# Autodesk Inventor assembly: 000-base_wheel-v1
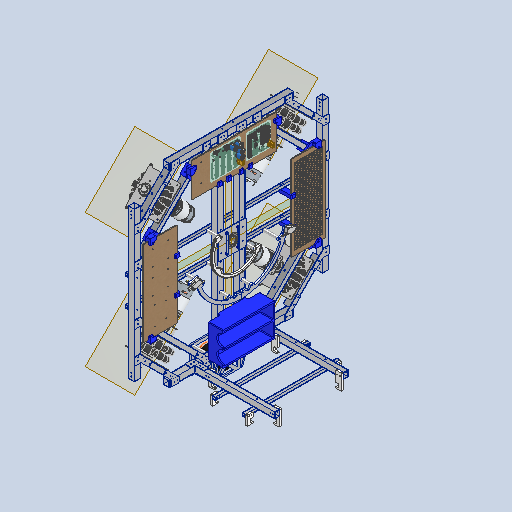
[picture p0: Inventor's stored thumbnail of the model, 512x512]
Saved by Autodesk Inventor 2025.2 (Build 292293000, 293)
## iProperties
Created: 2025-01-06
Part Number: 000-base_wheel-v1
Document SubType Name: Assembly
Designer: haruy
Mass: 4431.15 g
Surface Area: 15153.5 cm^2
Volume: 1600.59 cm^3
Density: 2.76846 g/cm^3
Author: haruy
## Documents named in this file (72)
- C:\Users\haruy\Documents\ロボコン\NHK2025\cad\nagahisa\base_weel\000-base_wheel-v1.iam
- C:\Users\haruy\Documents\ロボコン\NHK2025\cad\nagahisa\base_weel\base_weel-v2-ASP-Base.ipt
- C:\Users\haruy\Documents\ロボコン\NHK2025\cad\nagahisa\base_weel\base_weel-v2-Plate-1.ipt
- C:\Users\haruy\Documents\ロボコン\NHK2025\cad\nagahisa\base_weel\C-FL6904ZZ.ipt
- C:\Users\haruy\Documents\ロボコン\NHK2025\cad\nagahisa\base_weel\base_weel-v1-Shaft-spesa-1.ipt
- C:\Users\haruy\Documents\ロボコン\NHK2025\cad\nagahisa\base_weel\base_weel-v2-Plate-2.ipt
- C:\Users\haruy\Documents\ロボコン\NHK2025\cad\nagahisa\base_weel\takagi_weel\Workspaces\作業スペース\takagi\omuni_wheel_ver3.0\parts\omu_al_jo_1.ipt
- C:\Users\haruy\Documents\ロボコン\NHK2025\cad\nagahisa\base_weel\takagi_weel\Workspaces\作業スペース\takagi\omuni_wheel_ver3.0\parts\omu_al_jo_3.ipt
- C:\Users\haruy\Documents\ロボコン\NHK2025\cad\nagahisa\base_weel\takagi_weel\Workspaces\作業スペース\takagi\omuni_wheel_ver3.0\parts\frequently used parts\モーター\RS775\rs775_4.iam
- C:\Users\haruy\Documents\ロボコン\NHK2025\cad\nagahisa\base_weel\takagi_weel\Workspaces\作業スペース\takagi\omuni_wheel_ver3.0\parts\frequently used parts\セットカラー\SSCSP12-10\SSCSP12-10.iam
- C:\Users\haruy\Documents\ロボコン\NHK2025\cad\nagahisa\base_weel\takagi_weel\Workspaces\作業スペース\takagi\omuni_wheel_ver3.0\parts\omu_al_jo_2.ipt
- C:\Users\haruy\Documents\ロボコン\NHK2025\cad\nagahisa\base_weel\takagi_weel\Workspaces\作業スペース\takagi\omuni_wheel_ver3.0\parts\omu_sh_jo_2.ipt
- C:\Users\haruy\Documents\ロボコン\NHK2025\cad\nagahisa\base_weel\takagi_weel\Workspaces\作業スペース\takagi\omuni_wheel_ver3.0\parts\omu_sh_jo_3.ipt
- C:\Users\haruy\Documents\ロボコン\NHK2025\cad\nagahisa\base_weel\takagi_weel\Workspaces\作業スペース\takagi\omuni_wheel_ver3.0\parts\frequently used parts\ベアリング\B6201ZZNR\bearingB6201ZZNR.ipt
- C:\Users\haruy\Documents\ロボコン\NHK2025\cad\nagahisa\base_weel\takagi_weel\Workspaces\作業スペース\takagi\omuni_wheel_ver3.0\parts\frequently used parts\タイヤ\omni wheel\100mm wheel\100mm omuniwheel_MIR1.iam
- C:\Users\haruy\Documents\ロボコン\NHK2025\cad\nagahisa\base_weel\base_weel-v1-Shaft-spesa-2.ipt
- C:\Users\haruy\Documents\ロボコン\NHK2025\cad\nagahisa\base_weel\000-base_wheel-v1\デザイン アクセラレータ\平歯車1.iam
- C:\Users\haruy\Documents\ロボコン\NHK2025\cad\nagahisa\base_weel\base_weel-v1-Shaft-spesa-3.ipt
- C:\Users\haruy\Documents\ロボコン\NHK2025\cad\nagahisa\base_weel\takagi_weel\Workspaces\作業スペース\takagi\omuni_wheel_ver3.0\parts\omu_al_jo_1_MIR2.ipt
- C:\Users\haruy\Documents\ロボコン\NHK2025\cad\nagahisa\base_weel\takagi_weel\Workspaces\作業スペース\takagi\omuni_wheel_ver3.0\parts\omu_al_jo_3_MIR2.ipt
- C:\Users\haruy\Documents\ロボコン\NHK2025\cad\nagahisa\base_weel\takagi_weel\Workspaces\作業スペース\takagi\omuni_wheel_ver3.0\parts\frequently used parts\モーター\RS775\rs775_4_MIR2.iam
- C:\Users\haruy\Documents\ロボコン\NHK2025\cad\nagahisa\base_weel\takagi_weel\Workspaces\作業スペース\takagi\omuni_wheel_ver3.0\parts\frequently used parts\セットカラー\SSCSP12-10\SSCSP12-10_MIR2.iam
- C:\Users\haruy\Documents\ロボコン\NHK2025\cad\nagahisa\base_weel\takagi_weel\Workspaces\作業スペース\takagi\omuni_wheel_ver3.0\parts\omu_al_jo_2_MIR2.ipt
- C:\Users\haruy\Documents\ロボコン\NHK2025\cad\nagahisa\base_weel\takagi_weel\Workspaces\作業スペース\takagi\omuni_wheel_ver3.0\parts\omu_sh_jo_2_MIR2.ipt
- C:\Users\haruy\Documents\ロボコン\NHK2025\cad\nagahisa\base_weel\takagi_weel\Workspaces\作業スペース\takagi\omuni_wheel_ver3.0\parts\omu_sh_jo_3_MIR2.ipt
- C:\Users\haruy\Documents\ロボコン\NHK2025\cad\nagahisa\base_weel\takagi_weel\Workspaces\作業スペース\takagi\omuni_wheel_ver3.0\parts\frequently used parts\ベアリング\B6201ZZNR\bearingB6201ZZNR_MIR2.ipt
- C:\Users\haruy\Documents\ロボコン\NHK2025\cad\nagahisa\base_weel\takagi_weel\Workspaces\作業スペース\takagi\omuni_wheel_ver3.0\parts\frequently used parts\タイヤ\omni wheel\100mm wheel\100mm omuniwheel_MIR1_MIR.iam
- C:\Users\haruy\Documents\ロボコン\NHK2025\cad\nagahisa\base_weel\takagi_weel\Workspaces\作業スペース\takagi\omuni_wheel_ver3.0\parts\omu_al_jo_1_MIR3.ipt
- C:\Users\haruy\Documents\ロボコン\NHK2025\cad\nagahisa\base_weel\takagi_weel\Workspaces\作業スペース\takagi\omuni_wheel_ver3.0\parts\omu_al_jo_3_MIR3.ipt
- C:\Users\haruy\Documents\ロボコン\NHK2025\cad\nagahisa\base_weel\takagi_weel\Workspaces\作業スペース\takagi\omuni_wheel_ver3.0\parts\frequently used parts\モーター\RS775\rs775_4_MIR3.iam
- C:\Users\haruy\Documents\ロボコン\NHK2025\cad\nagahisa\base_weel\takagi_weel\Workspaces\作業スペース\takagi\omuni_wheel_ver3.0\parts\frequently used parts\セットカラー\SSCSP12-10\SSCSP12-10_MIR3.iam
- C:\Users\haruy\Documents\ロボコン\NHK2025\cad\nagahisa\base_weel\takagi_weel\Workspaces\作業スペース\takagi\omuni_wheel_ver3.0\parts\omu_al_jo_2_MIR3.ipt
- C:\Users\haruy\Documents\ロボコン\NHK2025\cad\nagahisa\base_weel\takagi_weel\Workspaces\作業スペース\takagi\omuni_wheel_ver3.0\parts\omu_sh_jo_2_MIR3.ipt
- C:\Users\haruy\Documents\ロボコン\NHK2025\cad\nagahisa\base_weel\takagi_weel\Workspaces\作業スペース\takagi\omuni_wheel_ver3.0\parts\omu_sh_jo_3_MIR3.ipt
- C:\Users\haruy\Documents\ロボコン\NHK2025\cad\nagahisa\base_weel\takagi_weel\Workspaces\作業スペース\takagi\omuni_wheel_ver3.0\parts\frequently used parts\ベアリング\B6201ZZNR\bearingB6201ZZNR_MIR3.ipt
- C:\Users\haruy\Documents\ロボコン\NHK2025\cad\nagahisa\base_weel\takagi_weel\Workspaces\作業スペース\takagi\omuni_wheel_ver3.0\parts\frequently used parts\タイヤ\omni wheel\100mm wheel\100mm omuniwheel_MIR1_MIR1.iam
- C:\Users\haruy\Documents\ロボコン\NHK2025\cad\nagahisa\base_weel\takagi_weel\Workspaces\作業スペース\takagi\omuni_wheel_ver3.0\parts\omu_al_jo_1_MIR2_MIR.ipt
- C:\Users\haruy\Documents\ロボコン\NHK2025\cad\nagahisa\base_weel\takagi_weel\Workspaces\作業スペース\takagi\omuni_wheel_ver3.0\parts\omu_al_jo_3_MIR2_MIR.ipt
- C:\Users\haruy\Documents\ロボコン\NHK2025\cad\nagahisa\base_weel\takagi_weel\Workspaces\作業スペース\takagi\omuni_wheel_ver3.0\parts\frequently used parts\モーター\RS775\rs775_4_MIR2_MIR.iam
- C:\Users\haruy\Documents\ロボコン\NHK2025\cad\nagahisa\base_weel\takagi_weel\Workspaces\作業スペース\takagi\omuni_wheel_ver3.0\parts\frequently used parts\セットカラー\SSCSP12-10\SSCSP12-10_MIR2_MIR.iam
- C:\Users\haruy\Documents\ロボコン\NHK2025\cad\nagahisa\base_weel\takagi_weel\Workspaces\作業スペース\takagi\omuni_wheel_ver3.0\parts\omu_al_jo_2_MIR2_MIR.ipt
- C:\Users\haruy\Documents\ロボコン\NHK2025\cad\nagahisa\base_weel\takagi_weel\Workspaces\作業スペース\takagi\omuni_wheel_ver3.0\parts\omu_sh_jo_2_MIR2_MIR.ipt
- C:\Users\haruy\Documents\ロボコン\NHK2025\cad\nagahisa\base_weel\takagi_weel\Workspaces\作業スペース\takagi\omuni_wheel_ver3.0\parts\omu_sh_jo_3_MIR2_MIR.ipt
- C:\Users\haruy\Documents\ロボコン\NHK2025\cad\nagahisa\base_weel\takagi_weel\Workspaces\作業スペース\takagi\omuni_wheel_ver3.0\parts\frequently used parts\ベアリング\B6201ZZNR\bearingB6201ZZNR_MIR2_MIR.ipt
- C:\Users\haruy\Documents\ロボコン\NHK2025\cad\nagahisa\base_weel\takagi_weel\Workspaces\作業スペース\takagi\omuni_wheel_ver3.0\parts\frequently used parts\タイヤ\omni wheel\100mm wheel\100mm omuniwheel_MIR1_MIR_MIR.iam
- C:\Users\haruy\Documents\ロボコン\NHK2025\cad\nagahisa\base_weel\base_weel-v2-Plate-3.ipt
- C:\Users\haruy\Documents\ロボコン\NHK2025\cad\nagahisa\base_weel\base_weel-v2-Plate-3_MIR.ipt
- C:\Users\haruy\Documents\ロボコン\NHK2025\cad\nagahisa\base_weel\base_weel-v2-Plate-3_MIR1.ipt
- C:\Users\haruy\Documents\ロボコン\NHK2025\cad\nagahisa\base_weel\base_weel-v2-Plate-3_MIR_MIR.ipt
- C:\Users\haruy\Documents\ロボコン\NHK2025\cad\nagahisa\base_weel\base_weel-v2-Plate-4.ipt
- C:\Users\haruy\Documents\ロボコン\NHK2025\cad\nagahisa\base_weel\base_weel-v2-Plate-5.ipt
- C:\Users\haruy\Documents\ロボコン\NHK2025\cad\000_parts\センサー\LiDAR_true.iam
- C:\Users\haruy\Documents\ロボコン\NHK2025\cad\nagahisa\base_weel\base_weel-v1-Shaft-lider-spesa.ipt
- C:\Users\haruy\Documents\ロボコン\NHK2025\cad\nagahisa\base_weel\base_weel-v2-Plate-6.ipt
- C:\Users\haruy\Documents\ロボコン\NHK2025\cad\nagahisa\base_weel\base_weel-v2-Plate-7.ipt
- C:\Users\haruy\Documents\ロボコン\NHK2025\cad\nagahisa\base_weel\base_weel-v2-3DP-C-F-1.ipt
- C:\Users\haruy\Documents\ロボコン\NHK2025\cad\nagahisa\base_weel\base_weel-v2-3DP-C-F-1_MIR.ipt
- C:\Users\haruy\Documents\ロボコン\NHK2025\cad\nagahisa\base_weel\base_weel-v2-MDF-1.ipt
- C:\Users\haruy\Documents\ロボコン\NHK2025\cad\000_parts\回路関連\DCMD_Controller.ipt
- C:\Users\haruy\Documents\ロボコン\NHK2025\cad\000_parts\回路関連\mbed_Board.ipt
- C:\Users\haruy\Documents\ロボコン\NHK2025\cad\nagahisa\base_weel\base_weel-v2-MDF-2.ipt
- C:\Users\haruy\Documents\ロボコン\NHK2025\cad\nagahisa\base_weel\roja-v1-3DP-lipo-box.ipt
- C:\Users\haruy\Documents\ロボコン\NHK2025\cad\nagahisa\base_weel\base_weel-v2-Plate-8.ipt
- C:\Users\haruy\Documents\ロボコン\NHK2025\cad\nagahisa\base_weel\base_weel-v2-POM-pc-F-1.ipt
- C:\Users\haruy\Documents\ロボコン\NHK2025\cad\nagahisa\base_weel\base_weel-v2-POM-pc-F-2.ipt
- C:\Users\haruy\Documents\ロボコン\NHK2025\cad\nagahisa\base_weel\base_weel-v2-MDF-3.ipt
- C:\Users\haruy\Documents\ロボコン\NHK2025\cad\000_parts\センサー\VX-012-1A3\VX-012-1A3\VX-012-1A3.iam
- C:\Users\haruy\Documents\ロボコン\NHK2025\cad\nagahisa\base_weel\base_weel-v2-3DP-C-F-2.ipt
- C:\Users\haruy\Documents\ロボコン\NHK2025\cad\nagahisa\base_weel\base_weel-v2-3DP-C-F-3.ipt
- C:\Users\haruy\Documents\ロボコン\NHK2025\cad\nagahisa\base_weel\base_weel-v2-Plate-9.ipt
- C:\Users\haruy\Documents\ロボコン\NHK2025\cad\nagahisa\base_weel\base_weel-v2-3DP-spesa-1.ipt
- C:\Users\haruy\Documents\ロボコン\NHK2025\cad\nagahisa\base_weel\base_weel-v2-Plate-10.ipt
## Components (133 placed, 71 different names)
1. base_weel-v2-ASP-Base:1 — 挿入:8, 挿入:9, 挿入:12, 挿入:13, 角度:1, 挿入:29, フラッシュ:1, 挿入:30, 挿入:32, 挿入:35, 挿入:36, 挿入:48, 挿入:49, 挿入:50, 挿入:51, 挿入:74, 挿入:75, 挿入:76, 挿入:77, 挿入:78, 挿入:79, 挿入:80, 挿入:81, 挿入:82, 挿入:83, 挿入:84, 挿入:85, 挿入:86, 挿入:87, 挿入:88, 挿入:89, 挿入:90, 挿入:91, 挿入:92, 挿入:93, 挿入:94, 挿入:95, 挿入:96, 挿入:97, 挿入:98, 挿入:99, 挿入:100, 挿入:101, 挿入:102, 挿入:103, 挿入:104, 挿入:105, 挿入:106, 挿入:107, 挿入:108, 挿入:109, 挿入:110, 挿入:111, 挿入:112, 挿入:113, 挿入:114, 挿入:115, 挿入:116, 挿入:117, 挿入:118, 挿入:119, 挿入:120, 挿入:121, 挿入:122, フラッシュ:2, 挿入:129, 挿入:130, 角度:4, 角度:5, 角度:6, 挿入:149, 挿入:151, 挿入:152, 挿入:153, 挿入:154, 挿入:155, 挿入:156, 挿入:157, 挿入:158, 挿入:159, 挿入:160, 挿入:161, 挿入:162, 挿入:163, 挿入:164, 挿入:165, 挿入:166, 挿入:167, 挿入:168, 挿入:169, 挿入:170, 挿入:171, 挿入:172, 挿入:173, 挿入:174, 挿入:185, 挿入:186, 挿入:187, 挿入:188, 挿入:189, 挿入:190, 挿入:191, 挿入:192, 挿入:193, 挿入:194, 挿入:195, 挿入:196, 挿入:197, 挿入:198, 挿入:199, 挿入:200, 挿入:201, 挿入:202, メイト:19, 挿入:203, 挿入:204, メイト:20, 挿入:205, 挿入:206, メイト:21, 挿入:216, 挿入:217, 挿入:218
2. base_weel-v2-Plate-1:1 — 挿入:3, 挿入:217, 挿入:218, 挿入:219, 挿入:220, 挿入:221, 挿入:222
3. C-FL6904ZZ:1 — 挿入:3, メイト:5
4. base_weel-v2-Plate-2:1 — 挿入:27, 挿入:207, 挿入:208, 挿入:209, 挿入:215
5. base_weel-v1-Shaft-spesa-1:3 — 挿入:8, 挿入:210
6. base_weel-v1-Shaft-spesa-1:4 — 挿入:9, 挿入:209
7. omu_al_jo_1:1 — 挿入:20, 挿入:21, 挿入:23, 挿入:35, 挿入:36
8. omu_al_jo_3:1 — 挿入:12, 挿入:13, 挿入:22
9. rs775_4:1 [sub-assembly]
10. SSCSP12-10:1 [sub-assembly]
11. omu_al_jo_2:1
12. omu_sh_jo_2:1
13. omu_sh_jo_3:1 — 挿入:21
14. omu_sh_jo_3:2
15. omu_sh_jo_3:3 — 挿入:20
16. omu_sh_jo_3:4
17. bearingB6201ZZNR:1 — 挿入:23, 挿入:24
18. bearingB6201ZZNR:2 — 挿入:22
19. 100mm omuniwheel_MIR1:1 [sub-assembly] — 角度:1, 挿入:24
20. base_weel-v1-Shaft-spesa-2:1 — 挿入:30, 挿入:211
21. base_weel-v1-Shaft-spesa-2:2 — 挿入:27, 挿入:29
22. 平歯車:1 [sub-assembly] — メイト:5, メイト:6, 挿入:31, 挿入:33, 挿入:34
23. base_weel-v1-Shaft-spesa-3:1 — 挿入:31, 挿入:32
24. base_weel-v1-Shaft-spesa-3:2 — 挿入:33
25. base_weel-v1-Shaft-spesa-3:3 — 挿入:34
26. omu_al_jo_1_MIR2:1 — 挿入:39, 挿入:42, 挿入:45, 挿入:50, 挿入:51
27. omu_al_jo_3_MIR2:1 — 挿入:46, 挿入:48, 挿入:49
28. rs775_4_MIR2:1 [sub-assembly] — メイト:7, 挿入:37, 挿入:38, メイト:8, メイト:9
29. SSCSP12-10_MIR2:1 [sub-assembly] — メイト:7, メイト:10
30. omu_al_jo_2_MIR2:1 — 挿入:37, 挿入:38, 挿入:40, 挿入:41, 挿入:43, 挿入:44
31. omu_sh_jo_2_MIR2:1 — メイト:8, メイト:9, メイト:10
32. omu_sh_jo_3_MIR2:1 — 挿入:39, 挿入:40
33. omu_sh_jo_3_MIR2:2 — 挿入:41
34. omu_sh_jo_3_MIR2:3 — 挿入:42, 挿入:43
35. omu_sh_jo_3_MIR2:4 — 挿入:44
36. bearingB6201ZZNR_MIR2:1 — 挿入:45, 挿入:47
37. bearingB6201ZZNR_MIR2:2 — 挿入:46
38. 100mm omuniwheel_MIR1_MIR:1 [sub-assembly] — 挿入:47, 角度:4
39. omu_al_jo_1_MIR3:1 — 挿入:54, 挿入:57, 挿入:60, 挿入:74, 挿入:75
40. omu_al_jo_3_MIR3:1 — 挿入:61, 挿入:76, 挿入:77
41. rs775_4_MIR3:1 [sub-assembly] — メイト:11, 挿入:52, 挿入:53, メイト:12, メイト:13
42. SSCSP12-10_MIR3:1 [sub-assembly] — メイト:11, メイト:14
43. omu_al_jo_2_MIR3:1 — 挿入:52, 挿入:53, 挿入:55, 挿入:56, 挿入:58, 挿入:59
44. omu_sh_jo_2_MIR3:1 — メイト:12, メイト:13, メイト:14
45. omu_sh_jo_3_MIR3:1 — 挿入:54, 挿入:55
46. omu_sh_jo_3_MIR3:2 — 挿入:56
47. omu_sh_jo_3_MIR3:3 — 挿入:57, 挿入:58
48. omu_sh_jo_3_MIR3:4 — 挿入:59
49. bearingB6201ZZNR_MIR3:1 — 挿入:60, 挿入:62
50. bearingB6201ZZNR_MIR3:2 — 挿入:61
51. 100mm omuniwheel_MIR1_MIR1:1 [sub-assembly] — 挿入:62, 角度:6
52. omu_al_jo_1_MIR2_MIR:1 — 挿入:66, 挿入:69, 挿入:71, 挿入:80, 挿入:81
53. omu_al_jo_3_MIR2_MIR:1 — 挿入:72, 挿入:78, 挿入:79
54. rs775_4_MIR2_MIR:1 [sub-assembly] — メイト:15, 挿入:63, 挿入:64, メイト:17, メイト:18
55. SSCSP12-10_MIR2_MIR:1 [sub-assembly] — メイト:15, メイト:16
56. omu_al_jo_2_MIR2_MIR:1 — 挿入:63, 挿入:64, 挿入:65, 挿入:67, 挿入:68, 挿入:70
57. omu_sh_jo_2_MIR2_MIR:1 — メイト:16, メイト:17, メイト:18
58. omu_sh_jo_3_MIR2_MIR:1 — 挿入:65, 挿入:66
59. omu_sh_jo_3_MIR2_MIR:2 — 挿入:67
60. omu_sh_jo_3_MIR2_MIR:3 — 挿入:68, 挿入:69
61. omu_sh_jo_3_MIR2_MIR:4 — 挿入:70
62. bearingB6201ZZNR_MIR2_MIR:1 — 挿入:71, 挿入:73
63. bearingB6201ZZNR_MIR2_MIR:2 — 挿入:72
64. 100mm omuniwheel_MIR1_MIR_MIR:1 [sub-assembly] — 挿入:73, 角度:5
65. base_weel-v2-Plate-3:1 — 挿入:82, 挿入:84
66. base_weel-v2-Plate-3:2 — 挿入:83, 挿入:85, 挿入:86
67. base_weel-v2-Plate-3:3 — 挿入:87, 挿入:88
68. base_weel-v2-Plate-3:4 — 挿入:89, 挿入:90
69. base_weel-v2-Plate-3_MIR:1 — 挿入:95, 挿入:96
70. base_weel-v2-Plate-3_MIR:2 — 挿入:97, 挿入:98
71. base_weel-v2-Plate-3_MIR:3 — 挿入:91, 挿入:92
72. base_weel-v2-Plate-3_MIR:4 — 挿入:93, 挿入:94
73. base_weel-v2-Plate-3_MIR1:1 — 挿入:101, 挿入:102
74. base_weel-v2-Plate-3_MIR1:2 — 挿入:99, 挿入:100
75. base_weel-v2-Plate-3_MIR1:3 — 挿入:103, 挿入:104
76. base_weel-v2-Plate-3_MIR1:4 — 挿入:105, 挿入:106
77. base_weel-v2-Plate-3_MIR_MIR:1 — 挿入:113, 挿入:114
78. base_weel-v2-Plate-3_MIR_MIR:2 — 挿入:111, 挿入:112
79. base_weel-v2-Plate-3_MIR_MIR:3 — 挿入:109, 挿入:110
80. base_weel-v2-Plate-3_MIR_MIR:4 — 挿入:107, 挿入:108
81. base_weel-v2-Plate-4:1 — 挿入:116, 挿入:117
82. base_weel-v2-Plate-4:2 — 挿入:115, 挿入:118
83. base_weel-v2-Plate-4:3 — 挿入:121, 挿入:122
84. base_weel-v2-Plate-4:4 — 挿入:119, 挿入:120
85. base_weel-v2-Plate-5:1 — 挿入:123, 挿入:124, フラッシュ:2, 挿入:125, 挿入:126, 角度:2, 角度:3, 挿入:131, 挿入:132
86. LiDAR_true:1 [sub-assembly] — 挿入:123, 挿入:124
87. base_weel-v1-Shaft-lider-spesa:1 — 挿入:126, 挿入:128
88. base_weel-v1-Shaft-lider-spesa:2 — 挿入:125, 挿入:127
89. base_weel-v2-Plate-6:1 — 挿入:127, 挿入:128
90. base_weel-v2-Plate-7:1 — 挿入:129, 角度:2, 挿入:131, 挿入:132
91. base_weel-v2-Plate-7:2 — 挿入:130, 角度:3
92. base_weel-v2-3DP-C-F-1:1 — 挿入:138, 挿入:201, 挿入:202
93. base_weel-v2-3DP-C-F-1_MIR:1 — 挿入:137, メイト:19
94. base_weel-v2-MDF-1:1 — 挿入:137, 挿入:138, 挿入:139, 挿入:140, 挿入:141, 挿入:142
95. DCMD_Controller:1 — 挿入:141, 挿入:142
96. mbed_Board:1 — 挿入:139, 挿入:140
97. base_weel-v2-3DP-C-F-1:2 — 挿入:148, 挿入:203, 挿入:204
98. base_weel-v2-3DP-C-F-1_MIR:2 — 挿入:147, メイト:20
99. base_weel-v2-MDF-2:1 — 挿入:147, 挿入:148
100. roja-v1-3DP-lipo-box:1 — 挿入:149, 挿入:216
101. base_weel-v2-Plate-8:1 — 挿入:151, 挿入:152
102. base_weel-v2-Plate-8:2 — 挿入:153, 挿入:154
103. base_weel-v2-Plate-8:3 — 挿入:155, 挿入:156
104. base_weel-v2-Plate-8:4 — 挿入:157, 挿入:158
105. base_weel-v2-POM-pc-F-1:1 — 挿入:159, 挿入:160
106. base_weel-v2-POM-pc-F-1:2 — 挿入:165, 挿入:166
107. base_weel-v2-POM-pc-F-1:3 — 挿入:161, 挿入:162
108. base_weel-v2-POM-pc-F-1:4 — 挿入:163, 挿入:164
109. base_weel-v2-POM-pc-F-2:1 — 挿入:169, 挿入:170
110. base_weel-v2-POM-pc-F-2:2 — 挿入:167, 挿入:168
111. base_weel-v2-POM-pc-F-2:3 — 挿入:173, 挿入:174
112. base_weel-v2-POM-pc-F-2:4 — 挿入:171, 挿入:172
113. base_weel-v2-3DP-C-F-1:3 — 挿入:179, 挿入:205, 挿入:206
114. base_weel-v2-3DP-C-F-1_MIR:3 — 挿入:180, メイト:21
115. base_weel-v2-MDF-3:1 — 挿入:179, 挿入:180
116. VX-012-1A3:1 [sub-assembly] — 挿入:212, 挿入:213
117. VX-012-1A3:2 [sub-assembly] — 挿入:207, 挿入:208
118. base_weel-v2-3DP-C-F-2:1 — 挿入:185, 挿入:186
119. base_weel-v2-3DP-C-F-2:2 — 挿入:187, 挿入:188
120. base_weel-v2-3DP-C-F-2:3 — 挿入:189, 挿入:190
121. base_weel-v2-3DP-C-F-2:4 — 挿入:191, 挿入:192
122. base_weel-v2-3DP-C-F-3:1 — 挿入:193, 挿入:194
123. base_weel-v2-3DP-C-F-3:2 — 挿入:195, 挿入:196
124. base_weel-v2-3DP-C-F-3:3 — 挿入:199, 挿入:200
125. base_weel-v2-3DP-C-F-3:4 — 挿入:197, 挿入:198
126. base_weel-v2-Plate-2:2 — 挿入:210, 挿入:211, 挿入:212, 挿入:213, 挿入:214
127. base_weel-v2-Plate-9:1 — 挿入:214, 挿入:215
128. base_weel-v2-3DP-spesa-1:1 — 挿入:219, 挿入:223
129. base_weel-v2-3DP-spesa-1:2 — 挿入:220, 挿入:224
130. base_weel-v2-3DP-spesa-1:3 — 挿入:222, 挿入:225
131. base_weel-v2-3DP-spesa-1:4 — 挿入:221, 挿入:226
132. base_weel-v2-Plate-10:1 — 挿入:223, 挿入:224
133. base_weel-v2-Plate-10:2 — 挿入:225, 挿入:226
## Relationships (227: Insert 198, Mate 21, Angle 6, Flush 2)
- 挿入:3 [Insert]: base_weel-v2-Plate-1:1 ↔ C-FL6904ZZ:1
- 挿入:8 [Insert]: base_weel-v2-ASP-Base:1 ↔ base_weel-v1-Shaft-spesa-1:3
- 挿入:9 [Insert]: base_weel-v2-ASP-Base:1 ↔ base_weel-v1-Shaft-spesa-1:4
- 挿入:12 [Insert]: base_weel-v2-ASP-Base:1 ↔ omu_al_jo_3:1
- 挿入:13 [Insert]: base_weel-v2-ASP-Base:1 ↔ omu_al_jo_3:1
- [Mate] (5 mm): rs775_4:1 ↔ SSCSP12-10:1
- [Insert]: rs775_4:1 ↔ omu_al_jo_2:1
- [Insert]: rs775_4:1 ↔ omu_al_jo_2:1
- [Mate]: SSCSP12-10:1 ↔ omu_sh_jo_2:1
- [Mate]: rs775_4:1 ↔ omu_sh_jo_2:1
- [Mate]: rs775_4:1 ↔ omu_sh_jo_2:1
- [Insert]: omu_al_jo_2:1 ↔ omu_sh_jo_3:1
- [Insert]: omu_al_jo_2:1 ↔ omu_sh_jo_3:4
- [Insert]: omu_al_jo_2:1 ↔ omu_sh_jo_3:2
- [Insert]: omu_al_jo_2:1 ↔ omu_sh_jo_3:3
- 挿入:20 [Insert]: omu_al_jo_1:1 ↔ omu_sh_jo_3:3
- 挿入:21 [Insert]: omu_al_jo_1:1 ↔ omu_sh_jo_3:1
- 挿入:22 [Insert]: omu_al_jo_3:1 ↔ bearingB6201ZZNR:2
- 挿入:23 [Insert]: omu_al_jo_1:1 ↔ bearingB6201ZZNR:1
- 角度:1 [Angle] (0 deg): base_weel-v2-ASP-Base:1 ↔ 100mm omuniwheel_MIR1:1
- 挿入:24 [Insert] (12 mm): bearingB6201ZZNR:1 ↔ 100mm omuniwheel_MIR1:1
- 挿入:27 [Insert]: base_weel-v2-Plate-2:1 ↔ base_weel-v1-Shaft-spesa-2:2
- 挿入:29 [Insert]: base_weel-v2-ASP-Base:1 ↔ base_weel-v1-Shaft-spesa-2:2
- フラッシュ:1 [Flush] (17 mm): base_weel-v2-ASP-Base:1
- 挿入:30 [Insert]: base_weel-v2-ASP-Base:1 ↔ base_weel-v1-Shaft-spesa-2:1
- メイト:5 [Mate]: C-FL6904ZZ:1 ↔ 平歯車:1
- メイト:6 [Mate]: 平歯車:1
- 挿入:31 [Insert]: 平歯車:1 ↔ base_weel-v1-Shaft-spesa-3:1
- 挿入:32 [Insert]: base_weel-v2-ASP-Base:1 ↔ base_weel-v1-Shaft-spesa-3:1
- 挿入:33 [Insert]: 平歯車:1 ↔ base_weel-v1-Shaft-spesa-3:2
- 挿入:34 [Insert]: 平歯車:1 ↔ base_weel-v1-Shaft-spesa-3:3
- 挿入:35 [Insert]: base_weel-v2-ASP-Base:1 ↔ omu_al_jo_1:1
- 挿入:36 [Insert]: base_weel-v2-ASP-Base:1 ↔ omu_al_jo_1:1
- メイト:7 [Mate] (5 mm): rs775_4_MIR2:1 ↔ SSCSP12-10_MIR2:1
- 挿入:37 [Insert]: rs775_4_MIR2:1 ↔ omu_al_jo_2_MIR2:1
- 挿入:38 [Insert]: rs775_4_MIR2:1 ↔ omu_al_jo_2_MIR2:1
- メイト:8 [Mate]: rs775_4_MIR2:1 ↔ omu_sh_jo_2_MIR2:1
- メイト:9 [Mate]: rs775_4_MIR2:1 ↔ omu_sh_jo_2_MIR2:1
- メイト:10 [Mate]: SSCSP12-10_MIR2:1 ↔ omu_sh_jo_2_MIR2:1
- 挿入:39 [Insert]: omu_al_jo_1_MIR2:1 ↔ omu_sh_jo_3_MIR2:1
- 挿入:40 [Insert]: omu_al_jo_2_MIR2:1 ↔ omu_sh_jo_3_MIR2:1
- 挿入:41 [Insert]: omu_al_jo_2_MIR2:1 ↔ omu_sh_jo_3_MIR2:2
- 挿入:42 [Insert]: omu_al_jo_1_MIR2:1 ↔ omu_sh_jo_3_MIR2:3
- 挿入:43 [Insert]: omu_al_jo_2_MIR2:1 ↔ omu_sh_jo_3_MIR2:3
- 挿入:44 [Insert]: omu_al_jo_2_MIR2:1 ↔ omu_sh_jo_3_MIR2:4
- 挿入:45 [Insert]: omu_al_jo_1_MIR2:1 ↔ bearingB6201ZZNR_MIR2:1
- 挿入:46 [Insert]: omu_al_jo_3_MIR2:1 ↔ bearingB6201ZZNR_MIR2:2
- 挿入:47 [Insert] (12 mm): bearingB6201ZZNR_MIR2:1 ↔ 100mm omuniwheel_MIR1_MIR:1
- 挿入:48 [Insert]: base_weel-v2-ASP-Base:1 ↔ omu_al_jo_3_MIR2:1
- 挿入:49 [Insert]: base_weel-v2-ASP-Base:1 ↔ omu_al_jo_3_MIR2:1
- 挿入:50 [Insert]: base_weel-v2-ASP-Base:1 ↔ omu_al_jo_1_MIR2:1
- 挿入:51 [Insert]: base_weel-v2-ASP-Base:1 ↔ omu_al_jo_1_MIR2:1
- メイト:11 [Mate] (5 mm): rs775_4_MIR3:1 ↔ SSCSP12-10_MIR3:1
- 挿入:52 [Insert]: rs775_4_MIR3:1 ↔ omu_al_jo_2_MIR3:1
- 挿入:53 [Insert]: rs775_4_MIR3:1 ↔ omu_al_jo_2_MIR3:1
- メイト:12 [Mate]: rs775_4_MIR3:1 ↔ omu_sh_jo_2_MIR3:1
- メイト:13 [Mate]: rs775_4_MIR3:1 ↔ omu_sh_jo_2_MIR3:1
- メイト:14 [Mate]: SSCSP12-10_MIR3:1 ↔ omu_sh_jo_2_MIR3:1
- 挿入:54 [Insert]: omu_al_jo_1_MIR3:1 ↔ omu_sh_jo_3_MIR3:1
- 挿入:55 [Insert]: omu_al_jo_2_MIR3:1 ↔ omu_sh_jo_3_MIR3:1
- 挿入:56 [Insert]: omu_al_jo_2_MIR3:1 ↔ omu_sh_jo_3_MIR3:2
- 挿入:57 [Insert]: omu_al_jo_1_MIR3:1 ↔ omu_sh_jo_3_MIR3:3
- 挿入:58 [Insert]: omu_al_jo_2_MIR3:1 ↔ omu_sh_jo_3_MIR3:3
- 挿入:59 [Insert]: omu_al_jo_2_MIR3:1 ↔ omu_sh_jo_3_MIR3:4
- 挿入:60 [Insert]: omu_al_jo_1_MIR3:1 ↔ bearingB6201ZZNR_MIR3:1
- 挿入:61 [Insert]: omu_al_jo_3_MIR3:1 ↔ bearingB6201ZZNR_MIR3:2
- 挿入:62 [Insert] (12 mm): bearingB6201ZZNR_MIR3:1 ↔ 100mm omuniwheel_MIR1_MIR1:1
- メイト:15 [Mate] (5 mm): rs775_4_MIR2_MIR:1 ↔ SSCSP12-10_MIR2_MIR:1
- 挿入:63 [Insert]: rs775_4_MIR2_MIR:1 ↔ omu_al_jo_2_MIR2_MIR:1
- 挿入:64 [Insert]: rs775_4_MIR2_MIR:1 ↔ omu_al_jo_2_MIR2_MIR:1
- メイト:16 [Mate]: SSCSP12-10_MIR2_MIR:1 ↔ omu_sh_jo_2_MIR2_MIR:1
- メイト:17 [Mate]: rs775_4_MIR2_MIR:1 ↔ omu_sh_jo_2_MIR2_MIR:1
- メイト:18 [Mate]: rs775_4_MIR2_MIR:1 ↔ omu_sh_jo_2_MIR2_MIR:1
- 挿入:65 [Insert]: omu_al_jo_2_MIR2_MIR:1 ↔ omu_sh_jo_3_MIR2_MIR:1
- 挿入:66 [Insert]: omu_al_jo_1_MIR2_MIR:1 ↔ omu_sh_jo_3_MIR2_MIR:1
- 挿入:67 [Insert]: omu_al_jo_2_MIR2_MIR:1 ↔ omu_sh_jo_3_MIR2_MIR:2
- 挿入:68 [Insert]: omu_al_jo_2_MIR2_MIR:1 ↔ omu_sh_jo_3_MIR2_MIR:3
- 挿入:69 [Insert]: omu_al_jo_1_MIR2_MIR:1 ↔ omu_sh_jo_3_MIR2_MIR:3
- 挿入:70 [Insert]: omu_al_jo_2_MIR2_MIR:1 ↔ omu_sh_jo_3_MIR2_MIR:4
- 挿入:71 [Insert]: omu_al_jo_1_MIR2_MIR:1 ↔ bearingB6201ZZNR_MIR2_MIR:1
- 挿入:72 [Insert]: omu_al_jo_3_MIR2_MIR:1 ↔ bearingB6201ZZNR_MIR2_MIR:2
- 挿入:73 [Insert] (12 mm): bearingB6201ZZNR_MIR2_MIR:1 ↔ 100mm omuniwheel_MIR1_MIR_MIR:1
- 挿入:74 [Insert]: base_weel-v2-ASP-Base:1 ↔ omu_al_jo_1_MIR3:1
- 挿入:75 [Insert]: base_weel-v2-ASP-Base:1 ↔ omu_al_jo_1_MIR3:1
- 挿入:76 [Insert]: base_weel-v2-ASP-Base:1 ↔ omu_al_jo_3_MIR3:1
- 挿入:77 [Insert]: base_weel-v2-ASP-Base:1 ↔ omu_al_jo_3_MIR3:1
- 挿入:78 [Insert]: base_weel-v2-ASP-Base:1 ↔ omu_al_jo_3_MIR2_MIR:1
- 挿入:79 [Insert]: base_weel-v2-ASP-Base:1 ↔ omu_al_jo_3_MIR2_MIR:1
- 挿入:80 [Insert]: base_weel-v2-ASP-Base:1 ↔ omu_al_jo_1_MIR2_MIR:1
- 挿入:81 [Insert]: base_weel-v2-ASP-Base:1 ↔ omu_al_jo_1_MIR2_MIR:1
- 挿入:82 [Insert]: base_weel-v2-ASP-Base:1 ↔ base_weel-v2-Plate-3:1
- 挿入:83 [Insert]: base_weel-v2-ASP-Base:1 ↔ base_weel-v2-Plate-3:2
- 挿入:84 [Insert]: base_weel-v2-ASP-Base:1 ↔ base_weel-v2-Plate-3:1
- 挿入:85 [Insert]: base_weel-v2-ASP-Base:1 ↔ base_weel-v2-Plate-3:2
- 挿入:86 [Insert]: base_weel-v2-ASP-Base:1 ↔ base_weel-v2-Plate-3:2
- 挿入:87 [Insert]: base_weel-v2-ASP-Base:1 ↔ base_weel-v2-Plate-3:3
- 挿入:88 [Insert]: base_weel-v2-ASP-Base:1 ↔ base_weel-v2-Plate-3:3
- 挿入:89 [Insert]: base_weel-v2-ASP-Base:1 ↔ base_weel-v2-Plate-3:4
- 挿入:90 [Insert]: base_weel-v2-ASP-Base:1 ↔ base_weel-v2-Plate-3:4
- 挿入:91 [Insert]: base_weel-v2-ASP-Base:1 ↔ base_weel-v2-Plate-3_MIR:3
- 挿入:92 [Insert]: base_weel-v2-ASP-Base:1 ↔ base_weel-v2-Plate-3_MIR:3
- 挿入:93 [Insert]: base_weel-v2-ASP-Base:1 ↔ base_weel-v2-Plate-3_MIR:4
- 挿入:94 [Insert]: base_weel-v2-ASP-Base:1 ↔ base_weel-v2-Plate-3_MIR:4
- 挿入:95 [Insert]: base_weel-v2-ASP-Base:1 ↔ base_weel-v2-Plate-3_MIR:1
- 挿入:96 [Insert]: base_weel-v2-ASP-Base:1 ↔ base_weel-v2-Plate-3_MIR:1
- 挿入:97 [Insert]: base_weel-v2-ASP-Base:1 ↔ base_weel-v2-Plate-3_MIR:2
- 挿入:98 [Insert]: base_weel-v2-ASP-Base:1 ↔ base_weel-v2-Plate-3_MIR:2
- 挿入:99 [Insert]: base_weel-v2-ASP-Base:1 ↔ base_weel-v2-Plate-3_MIR1:2
- 挿入:100 [Insert]: base_weel-v2-ASP-Base:1 ↔ base_weel-v2-Plate-3_MIR1:2
- 挿入:101 [Insert]: base_weel-v2-ASP-Base:1 ↔ base_weel-v2-Plate-3_MIR1:1
- 挿入:102 [Insert]: base_weel-v2-ASP-Base:1 ↔ base_weel-v2-Plate-3_MIR1:1
- 挿入:103 [Insert]: base_weel-v2-ASP-Base:1 ↔ base_weel-v2-Plate-3_MIR1:3
- 挿入:104 [Insert]: base_weel-v2-ASP-Base:1 ↔ base_weel-v2-Plate-3_MIR1:3
- 挿入:105 [Insert]: base_weel-v2-ASP-Base:1 ↔ base_weel-v2-Plate-3_MIR1:4
- 挿入:106 [Insert]: base_weel-v2-ASP-Base:1 ↔ base_weel-v2-Plate-3_MIR1:4
- 挿入:107 [Insert]: base_weel-v2-ASP-Base:1 ↔ base_weel-v2-Plate-3_MIR_MIR:4
- 挿入:108 [Insert]: base_weel-v2-ASP-Base:1 ↔ base_weel-v2-Plate-3_MIR_MIR:4
- 挿入:109 [Insert]: base_weel-v2-ASP-Base:1 ↔ base_weel-v2-Plate-3_MIR_MIR:3
- 挿入:110 [Insert]: base_weel-v2-ASP-Base:1 ↔ base_weel-v2-Plate-3_MIR_MIR:3
- 挿入:111 [Insert]: base_weel-v2-ASP-Base:1 ↔ base_weel-v2-Plate-3_MIR_MIR:2
- 挿入:112 [Insert]: base_weel-v2-ASP-Base:1 ↔ base_weel-v2-Plate-3_MIR_MIR:2
- 挿入:113 [Insert]: base_weel-v2-ASP-Base:1 ↔ base_weel-v2-Plate-3_MIR_MIR:1
- 挿入:114 [Insert]: base_weel-v2-ASP-Base:1 ↔ base_weel-v2-Plate-3_MIR_MIR:1
- 挿入:115 [Insert]: base_weel-v2-ASP-Base:1 ↔ base_weel-v2-Plate-4:2
- 挿入:116 [Insert]: base_weel-v2-ASP-Base:1 ↔ base_weel-v2-Plate-4:1
- 挿入:117 [Insert]: base_weel-v2-ASP-Base:1 ↔ base_weel-v2-Plate-4:1
- 挿入:118 [Insert]: base_weel-v2-ASP-Base:1 ↔ base_weel-v2-Plate-4:2
- 挿入:119 [Insert]: base_weel-v2-ASP-Base:1 ↔ base_weel-v2-Plate-4:4
- 挿入:120 [Insert]: base_weel-v2-ASP-Base:1 ↔ base_weel-v2-Plate-4:4
- 挿入:121 [Insert]: base_weel-v2-ASP-Base:1 ↔ base_weel-v2-Plate-4:3
- 挿入:122 [Insert]: base_weel-v2-ASP-Base:1 ↔ base_weel-v2-Plate-4:3
- 挿入:123 [Insert]: base_weel-v2-Plate-5:1 ↔ LiDAR_true:1
- 挿入:124 [Insert]: base_weel-v2-Plate-5:1 ↔ LiDAR_true:1
- フラッシュ:2 [Flush]: base_weel-v2-ASP-Base:1 ↔ base_weel-v2-Plate-5:1
- 挿入:125 [Insert]: base_weel-v2-Plate-5:1 ↔ base_weel-v1-Shaft-lider-spesa:2
- 挿入:126 [Insert]: base_weel-v2-Plate-5:1 ↔ base_weel-v1-Shaft-lider-spesa:1
- 挿入:127 [Insert]: base_weel-v1-Shaft-lider-spesa:2 ↔ base_weel-v2-Plate-6:1
- 挿入:128 [Insert]: base_weel-v1-Shaft-lider-spesa:1 ↔ base_weel-v2-Plate-6:1
- 挿入:129 [Insert]: base_weel-v2-ASP-Base:1 ↔ base_weel-v2-Plate-7:1
- 角度:2 [Angle] (0 deg): base_weel-v2-Plate-5:1 ↔ base_weel-v2-Plate-7:1
- 挿入:130 [Insert]: base_weel-v2-ASP-Base:1 ↔ base_weel-v2-Plate-7:2
- 角度:3 [Angle] (180 deg): base_weel-v2-Plate-5:1 ↔ base_weel-v2-Plate-7:2
- 挿入:131 [Insert]: base_weel-v2-Plate-5:1 ↔ base_weel-v2-Plate-7:1
- 挿入:132 [Insert]: base_weel-v2-Plate-5:1 ↔ base_weel-v2-Plate-7:1
- 角度:4 [Angle] (180 deg): base_weel-v2-ASP-Base:1 ↔ 100mm omuniwheel_MIR1_MIR:1
- 角度:5 [Angle] (180 deg): base_weel-v2-ASP-Base:1 ↔ 100mm omuniwheel_MIR1_MIR_MIR:1
- 角度:6 [Angle] (180 deg): base_weel-v2-ASP-Base:1 ↔ 100mm omuniwheel_MIR1_MIR1:1
- 挿入:137 [Insert]: base_weel-v2-3DP-C-F-1_MIR:1 ↔ base_weel-v2-MDF-1:1
- 挿入:138 [Insert]: base_weel-v2-3DP-C-F-1:1 ↔ base_weel-v2-MDF-1:1
- 挿入:139 [Insert]: base_weel-v2-MDF-1:1 ↔ mbed_Board:1
- 挿入:140 [Insert]: base_weel-v2-MDF-1:1 ↔ mbed_Board:1
- 挿入:141 [Insert]: base_weel-v2-MDF-1:1 ↔ DCMD_Controller:1
- 挿入:142 [Insert]: base_weel-v2-MDF-1:1 ↔ DCMD_Controller:1
- 挿入:147 [Insert]: base_weel-v2-3DP-C-F-1_MIR:2 ↔ base_weel-v2-MDF-2:1
- 挿入:148 [Insert]: base_weel-v2-3DP-C-F-1:2 ↔ base_weel-v2-MDF-2:1
- 挿入:149 [Insert]: base_weel-v2-ASP-Base:1 ↔ roja-v1-3DP-lipo-box:1
- 挿入:151 [Insert]: base_weel-v2-ASP-Base:1 ↔ base_weel-v2-Plate-8:1
- 挿入:152 [Insert]: base_weel-v2-ASP-Base:1 ↔ base_weel-v2-Plate-8:1
- 挿入:153 [Insert]: base_weel-v2-ASP-Base:1 ↔ base_weel-v2-Plate-8:2
- 挿入:154 [Insert]: base_weel-v2-ASP-Base:1 ↔ base_weel-v2-Plate-8:2
- 挿入:155 [Insert]: base_weel-v2-ASP-Base:1 ↔ base_weel-v2-Plate-8:3
- 挿入:156 [Insert]: base_weel-v2-ASP-Base:1 ↔ base_weel-v2-Plate-8:3
- 挿入:157 [Insert]: base_weel-v2-ASP-Base:1 ↔ base_weel-v2-Plate-8:4
- 挿入:158 [Insert]: base_weel-v2-ASP-Base:1 ↔ base_weel-v2-Plate-8:4
- 挿入:159 [Insert]: base_weel-v2-ASP-Base:1 ↔ base_weel-v2-POM-pc-F-1:1
- 挿入:160 [Insert]: base_weel-v2-ASP-Base:1 ↔ base_weel-v2-POM-pc-F-1:1
- 挿入:161 [Insert]: base_weel-v2-ASP-Base:1 ↔ base_weel-v2-POM-pc-F-1:3
- 挿入:162 [Insert]: base_weel-v2-ASP-Base:1 ↔ base_weel-v2-POM-pc-F-1:3
- 挿入:163 [Insert]: base_weel-v2-ASP-Base:1 ↔ base_weel-v2-POM-pc-F-1:4
- 挿入:164 [Insert]: base_weel-v2-ASP-Base:1 ↔ base_weel-v2-POM-pc-F-1:4
- 挿入:165 [Insert]: base_weel-v2-ASP-Base:1 ↔ base_weel-v2-POM-pc-F-1:2
- 挿入:166 [Insert]: base_weel-v2-ASP-Base:1 ↔ base_weel-v2-POM-pc-F-1:2
- 挿入:167 [Insert]: base_weel-v2-ASP-Base:1 ↔ base_weel-v2-POM-pc-F-2:2
- 挿入:168 [Insert]: base_weel-v2-ASP-Base:1 ↔ base_weel-v2-POM-pc-F-2:2
- 挿入:169 [Insert]: base_weel-v2-ASP-Base:1 ↔ base_weel-v2-POM-pc-F-2:1
- 挿入:170 [Insert]: base_weel-v2-ASP-Base:1 ↔ base_weel-v2-POM-pc-F-2:1
- 挿入:171 [Insert]: base_weel-v2-ASP-Base:1 ↔ base_weel-v2-POM-pc-F-2:4
- 挿入:172 [Insert]: base_weel-v2-ASP-Base:1 ↔ base_weel-v2-POM-pc-F-2:4
- 挿入:173 [Insert]: base_weel-v2-ASP-Base:1 ↔ base_weel-v2-POM-pc-F-2:3
- 挿入:174 [Insert]: base_weel-v2-ASP-Base:1 ↔ base_weel-v2-POM-pc-F-2:3
- 挿入:179 [Insert]: base_weel-v2-3DP-C-F-1:3 ↔ base_weel-v2-MDF-3:1
- 挿入:180 [Insert]: base_weel-v2-3DP-C-F-1_MIR:3 ↔ base_weel-v2-MDF-3:1
- 挿入:185 [Insert]: base_weel-v2-ASP-Base:1 ↔ base_weel-v2-3DP-C-F-2:1
- 挿入:186 [Insert]: base_weel-v2-ASP-Base:1 ↔ base_weel-v2-3DP-C-F-2:1
- 挿入:187 [Insert]: base_weel-v2-ASP-Base:1 ↔ base_weel-v2-3DP-C-F-2:2
- 挿入:188 [Insert]: base_weel-v2-ASP-Base:1 ↔ base_weel-v2-3DP-C-F-2:2
- 挿入:189 [Insert]: base_weel-v2-ASP-Base:1 ↔ base_weel-v2-3DP-C-F-2:3
- 挿入:190 [Insert]: base_weel-v2-ASP-Base:1 ↔ base_weel-v2-3DP-C-F-2:3
- 挿入:191 [Insert]: base_weel-v2-ASP-Base:1 ↔ base_weel-v2-3DP-C-F-2:4
- 挿入:192 [Insert]: base_weel-v2-ASP-Base:1 ↔ base_weel-v2-3DP-C-F-2:4
- 挿入:193 [Insert]: base_weel-v2-ASP-Base:1 ↔ base_weel-v2-3DP-C-F-3:1
- 挿入:194 [Insert]: base_weel-v2-ASP-Base:1 ↔ base_weel-v2-3DP-C-F-3:1
- 挿入:195 [Insert]: base_weel-v2-ASP-Base:1 ↔ base_weel-v2-3DP-C-F-3:2
- 挿入:196 [Insert]: base_weel-v2-ASP-Base:1 ↔ base_weel-v2-3DP-C-F-3:2
- 挿入:197 [Insert]: base_weel-v2-ASP-Base:1 ↔ base_weel-v2-3DP-C-F-3:4
- 挿入:198 [Insert]: base_weel-v2-ASP-Base:1 ↔ base_weel-v2-3DP-C-F-3:4
- 挿入:199 [Insert]: base_weel-v2-ASP-Base:1 ↔ base_weel-v2-3DP-C-F-3:3
- 挿入:200 [Insert]: base_weel-v2-ASP-Base:1 ↔ base_weel-v2-3DP-C-F-3:3
- 挿入:201 [Insert]: base_weel-v2-ASP-Base:1 ↔ base_weel-v2-3DP-C-F-1:1
- 挿入:202 [Insert]: base_weel-v2-ASP-Base:1 ↔ base_weel-v2-3DP-C-F-1:1
- メイト:19 [Mate] (0.2 mm): base_weel-v2-ASP-Base:1 ↔ base_weel-v2-3DP-C-F-1_MIR:1
- 挿入:203 [Insert]: base_weel-v2-ASP-Base:1 ↔ base_weel-v2-3DP-C-F-1:2
- 挿入:204 [Insert]: base_weel-v2-ASP-Base:1 ↔ base_weel-v2-3DP-C-F-1:2
- メイト:20 [Mate] (0.2 mm): base_weel-v2-ASP-Base:1 ↔ base_weel-v2-3DP-C-F-1_MIR:2
- 挿入:205 [Insert]: base_weel-v2-ASP-Base:1 ↔ base_weel-v2-3DP-C-F-1:3
- 挿入:206 [Insert]: base_weel-v2-ASP-Base:1 ↔ base_weel-v2-3DP-C-F-1:3
- メイト:21 [Mate]: base_weel-v2-ASP-Base:1 ↔ base_weel-v2-3DP-C-F-1_MIR:3
- 挿入:207 [Insert]: base_weel-v2-Plate-2:1 ↔ VX-012-1A3:2
- 挿入:208 [Insert]: base_weel-v2-Plate-2:1 ↔ VX-012-1A3:2
- 挿入:209 [Insert]: base_weel-v2-Plate-2:1 ↔ base_weel-v1-Shaft-spesa-1:4
- 挿入:210 [Insert]: base_weel-v1-Shaft-spesa-1:3 ↔ base_weel-v2-Plate-2:2
- 挿入:211 [Insert]: base_weel-v1-Shaft-spesa-2:1 ↔ base_weel-v2-Plate-2:2
- 挿入:212 [Insert]: VX-012-1A3:1 ↔ base_weel-v2-Plate-2:2
- 挿入:213 [Insert]: VX-012-1A3:1 ↔ base_weel-v2-Plate-2:2
- 挿入:214 [Insert]: base_weel-v2-Plate-2:2 ↔ base_weel-v2-Plate-9:1
- 挿入:215 [Insert]: base_weel-v2-Plate-2:1 ↔ base_weel-v2-Plate-9:1
- 挿入:216 [Insert]: base_weel-v2-ASP-Base:1 ↔ roja-v1-3DP-lipo-box:1
- 挿入:217 [Insert]: base_weel-v2-ASP-Base:1 ↔ base_weel-v2-Plate-1:1
- 挿入:218 [Insert]: base_weel-v2-ASP-Base:1 ↔ base_weel-v2-Plate-1:1
- 挿入:219 [Insert]: base_weel-v2-Plate-1:1 ↔ base_weel-v2-3DP-spesa-1:1
- 挿入:220 [Insert]: base_weel-v2-Plate-1:1 ↔ base_weel-v2-3DP-spesa-1:2
- 挿入:221 [Insert]: base_weel-v2-Plate-1:1 ↔ base_weel-v2-3DP-spesa-1:4
- 挿入:222 [Insert]: base_weel-v2-Plate-1:1 ↔ base_weel-v2-3DP-spesa-1:3
- 挿入:223 [Insert]: base_weel-v2-3DP-spesa-1:1 ↔ base_weel-v2-Plate-10:1
- 挿入:224 [Insert]: base_weel-v2-3DP-spesa-1:2 ↔ base_weel-v2-Plate-10:1
- 挿入:225 [Insert]: base_weel-v2-3DP-spesa-1:3 ↔ base_weel-v2-Plate-10:2
- 挿入:226 [Insert]: base_weel-v2-3DP-spesa-1:4 ↔ base_weel-v2-Plate-10:2
## Named parameters: d159_d51 = 0 mm, d160_d52 = 0 mm, d161_d53 = 0 mm, d165_d57 = 0 mm, d166_d58 = 0 mm, d167_d59 = 0 mm, d168_d60 = 0 mm, d176_d40 = 0 mm, d177_d41 = 0 mm, d178_d5 = 5 mm
